# Autodesk Inventor assembly: J005558
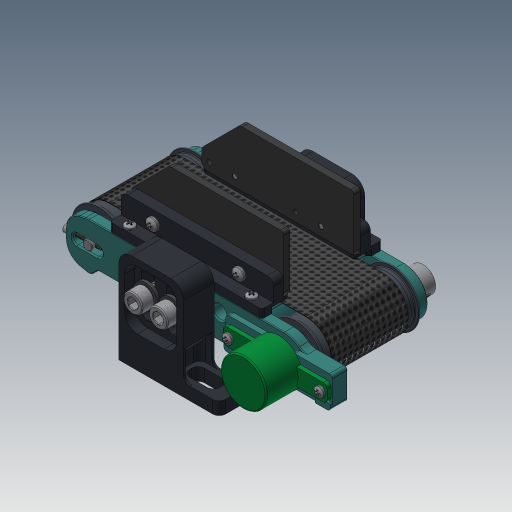
[picture p0: Inventor's stored thumbnail of the model, 512x512]
Saved by Autodesk Inventor 2023.3 (Build 273359000, 359)
## iProperties
Created: 2014-11-17
Vendor: HHMI: JRC - ID&F
Document SubType Name: Assembly
Designer: ARNOLDJ
Description: NRB TREADMILL ASSY
Project: COMMON
Part Number: J005558
RuleStatus: InUse
AfterDocSave0: file://Part Number Cleaner
DESIGN DEPARTMENT: HHMI: JRC - ID&F
LAB/DEPT: COMMON
REQUESTING SCIENTIST: COMMON
SPECIAL FINISH: N/A
SURFACE ROUGHNESS: N/A
ALTERED ITEM PART NUMBER: N/A
ALTERED ITEM VENDOR: N/A
ALTERED ITEM DESCRIPTION: N/A
Revision Number: 0
## Documents named in this file (27)
- C:\_WORKSPACE\DATA\PROJECTS\TREADMILLS\MOUSE NARROW RIBBON BELT TREADMILL\MCAD\NRB DRIVEN TREADMILL ASSY.iam
- C:\_WORKSPACE\DATA\PROJECTS\TREADMILLS\MOUSE MOTOR DRIVEN TREADMILL\MCAD\90107A126.ipt
- C:\_WORKSPACE\DATA\PROJECTS\TREADMILLS\MOUSE MOTOR DRIVEN TREADMILL\MCAD\57155K335.ipt
- C:\_WORKSPACE\DATA\PROJECTS\TREADMILLS\MOUSE MOTOR DRIVEN TREADMILL\MCAD\R233-05-5.ipt
- C:\_WORKSPACE\DATA\PROJECTS\TREADMILLS\MOUSE WIDE RIBBON BELT TREADMILL\MCAD\HEDR-5420-ES214.ipt
- C:\_WORKSPACE\DATA\PROJECTS\TREADMILLS\MOUSE NARROW RIBBON BELT TREADMILL\MCAD\NRB ROLLER.ipt
- C:\_WORKSPACE\DATA\PROJECTS\TREADMILLS\MOUSE NARROW RIBBON BELT TREADMILL\MCAD\NRB DRIVE ROLLER.ipt
- C:\_WORKSPACE\DATA\PROJECTS\TREADMILLS\MOUSE NARROW RIBBON BELT TREADMILL\MCAD\NRB IDLER SHAFT.ipt
- C:\_WORKSPACE\DATA\PROJECTS\TREADMILLS\MOUSE NARROW RIBBON BELT TREADMILL\MCAD\NRB DRIVE SHAFT.ipt
- C:\_WORKSPACE\DATA\PROJECTS\TREADMILLS\MOUSE NARROW RIBBON BELT TREADMILL\MCAD\98317A214.ipt
- C:\_WORKSPACE\DATA\PROJECTS\TREADMILLS\MOUSE NARROW RIBBON BELT TREADMILL\MCAD\57155K336.ipt
- C:\_WORKSPACE\DATA\PROJECTS\TREADMILLS\MOUSE NARROW RIBBON BELT TREADMILL\MCAD\9946K110.ipt
- C:\_WORKSPACE\DATA\PROJECTS\TREADMILLS\MOUSE NARROW RIBBON BELT TREADMILL\MCAD\NRB BRKT SIDE WALL.ipt
- C:\_WORKSPACE\DATA\PROJECTS\TREADMILLS\MOUSE NARROW RIBBON BELT TREADMILL\MCAD\92290A746.ipt
- C:\_WORKSPACE\DATA\PROJECTS\TREADMILLS\TREADMILL LEGO\MCAD\ROLLING WHEEL TYPE\90965A170.ipt
- C:\_WORKSPACE\DATA\PROJECTS\TREADMILLS\TREADMILL LEGO\MCAD\ROLLING WHEEL TYPE\92196A540.ipt
- C:\_WORKSPACE\DATA\PROJECTS\TREADMILLS\MOUSE NARROW RIBBON BELT TREADMILL\MCAD\NRB ADJ BRKT MR.ipt
- C:\_WORKSPACE\DATA\PROJECTS\TREADMILLS\MOUSE NARROW RIBBON BELT TREADMILL\MCAD\NRB ADJ BRKT ML.ipt
- C:\_WORKSPACE\DATA\PROJECTS\TREADMILLS\MOUSE NARROW RIBBON BELT TREADMILL\MCAD\NRB BELT.ipt
- C:\_WORKSPACE\DATA\PROJECTS\TREADMILLS\MOUSE NARROW RIBBON BELT TREADMILL\MCAD\92000A118.ipt
- C:\_WORKSPACE\DATA\PROJECTS\TREADMILLS\MOUSE NARROW RIBBON BELT TREADMILL\MCAD\NRB MAIN BODY INSERTS.ipt
- C:\_WORKSPACE\DATA\PROJECTS\TREADMILLS\MOUSE NARROW RIBBON BELT TREADMILL\MCAD\94785A415_TYPE 18-8 STAINLESS STEEL SQUARE NUT.ipt
- C:\_WORKSPACE\DATA\PROJECTS\TREADMILLS\MOUSE NARROW RIBBON BELT TREADMILL\MCAD\NRB LOW GUIDE RAIL INSERTS.ipt
- C:\_WORKSPACE\DATA\PROJECTS\TREADMILLS\MOUSE NARROW RIBBON BELT TREADMILL\MCAD\91828A113_TYPE 18-8 STAINLESS STEEL HEX NUT.ipt
- C:\_WORKSPACE\DATA\COMMON\McMaster\92000A106.ipt
- C:\_WORKSPACE\DATA\COMMON\McMaster\92000A112.ipt
- C:\_WORKSPACE\DATA\PROJECTS\TREADMILLS\MOUSE NARROW RIBBON BELT TREADMILL\MCAD\HEDR-5420-ES214_DISC.ipt
## Components (53 placed, 26 different names)
1. NRB MAIN BODY INSERTS:1 — Mate:11, Mate:12, Mate:78, Mate:79, Mate:80, Mate:81, Mate:97, Mate:99, Mate:124, Mate:125, Mate:126, Mate:127, Mate:179, Mate:180, Mate:181, Mate:185, Mate:186, Mate:187, Mate:211, Mate:212, Mate:213, Mate:214, Mate:215, Mate:216, Mate:217, Mate:218, Mate:219, Mate:220, Mate:221, Mate:222, Mate:223, Mate:224, Angle:7, Angle:8, Angle:9, Mate:225, Mate:226, Angle:10, Mate:227, Mate:228, Mate:229
2. 57155K336:2 — Mate:11, Mate:12, Mate:126, Mate:127
3. 57155K336:1 — Mate:124, Mate:125
4. NRB ROLLER:1 — Mate:18, Mate:19, Mate:35, Flush:5, Mate:54, Mate:55, Mate:56, Mate:57
5. 57155K335:7 — Mate:56, Mate:57
6. 57155K335:8 — Mate:54, Mate:55
7. NRB IDLER SHAFT:1 — Flush:2, Mate:35, Angle:5
8. NRB DRIVE SHAFT:1 — Mate:94, Mate:98, Mate:243, Flush:6
9. 9946K110:1
10. NRB DRIVE ROLLER:1 — Mate:60
11. NRB BELT:1 — Mate:62, Mate:63, Angle:6
12. 90107A126:1 — Mate:78, Mate:79
13. 90107A126:2 — Mate:80, Mate:81
14. 92290A746:1
15. 92290A746:2
16. R233-05-5:1
17. 98317A214:1
18. HEDR-5420-ES214:1 — Mate:97, Mate:98, Mate:99, Mate:231, Mate:232, Mate:241, Mate:242
19. 92196A540:3 — Mate:230
20. 90965A170:1
21. 92196A540:4
22. 90965A170:2
23. NRB ADJ BRKT ML:1
24. NRB ADJ BRKT MR:1
25. 92196A540:2
26. 90965A170:4
27. 92196A540:1
28. 90965A170:3
29. 92000A112:1 — Mate:233, Mate:234
30. 92000A112:2 — Mate:235, Mate:236
31. 92000A112:3 — Mate:237, Mate:238
32. 92000A112:4 — Mate:239, Mate:240
33. 92000A118:1 — Mate:193, Mate:194
34. 92000A118:2 — Mate:191, Mate:192
35. 92000A118:3 — Mate:207, Mate:208
36. 92000A118:4 — Mate:205, Mate:206
37. NRB LOW GUIDE RAIL INSERTS:1 — Mate:179, Mate:180, Mate:181, Mate:182, Mate:183, Mate:184, Mate:205, Mate:206, Mate:207, Mate:208, Mate:237, Mate:238, Mate:239, Mate:240
38. NRB BRKT SIDE WALL:2 — Mate:188, Mate:189, Mate:190, Mate:192
39. NRB BRKT SIDE WALL:3 — Mate:182, Mate:183, Mate:184
40. NRB LOW GUIDE RAIL INSERTS:2 — Mate:185, Mate:186, Mate:187, Mate:188, Mate:189, Mate:190, Mate:191, Mate:193, Mate:194, Mate:233, Mate:234, Mate:235, Mate:236
41. 94785A415_TYPE 18-8 STAINLESS STEEL SQUARE NUT:1 — Mate:211, Mate:212
42. 94785A415_TYPE 18-8 STAINLESS STEEL SQUARE NUT:2 — Mate:213, Mate:214
43. 91828A113_TYPE 18-8 STAINLESS STEEL HEX NUT:1 — Mate:215, Mate:216
44. 91828A113_TYPE 18-8 STAINLESS STEEL HEX NUT:2 — Mate:217, Mate:218
45. 91828A113_TYPE 18-8 STAINLESS STEEL HEX NUT:3 — Mate:219, Mate:220, Angle:8
46. 91828A113_TYPE 18-8 STAINLESS STEEL HEX NUT:4 — Mate:221, Mate:222, Angle:9
47. 91828A113_TYPE 18-8 STAINLESS STEEL HEX NUT:5 — Mate:223, Mate:224, Angle:7
48. 91828A113_TYPE 18-8 STAINLESS STEEL HEX NUT:6 — Mate:225, Mate:226, Angle:10
49. 94785A415_TYPE 18-8 STAINLESS STEEL SQUARE NUT:3 — Mate:227, Mate:228
50. 94785A415_TYPE 18-8 STAINLESS STEEL SQUARE NUT:4 — Mate:229, Mate:230
51. 92000A106:1 — Mate:231, Mate:232
52. 92000A112:5 — Mate:241, Mate:242
53. HEDR-5420-ES214_DISC:1 — Mate:243, Flush:6
## Relationships (129: Mate 119, Angle 6, Flush 4)
- Mate:11: NRB MAIN BODY INSERTS:1 ↔ 57155K336:2
- Mate:12: NRB MAIN BODY INSERTS:1 ↔ 57155K336:2
- Flush:1
- Mate:15
- Mate:16
- Mate:18: NRB ROLLER:1
- Mate:19: NRB ROLLER:1
- Flush:2: NRB IDLER SHAFT:1
- Mate:35: NRB ROLLER:1 ↔ NRB IDLER SHAFT:1
- Mate:94: NRB DRIVE SHAFT:1
- [Mate]: 57155K336:2 ↔ 9946K110:1
- [Mate]: NRB DRIVE SHAFT:1 ↔ 9946K110:1
- Flush:5: NRB ROLLER:1
- Mate:54: NRB ROLLER:1 ↔ 57155K335:8
- Mate:55: NRB ROLLER:1 ↔ 57155K335:8
- Mate:56: NRB ROLLER:1 ↔ 57155K335:7
- Mate:57: NRB ROLLER:1 ↔ 57155K335:7
- Angle:5 (0 deg): NRB IDLER SHAFT:1
- Mate:60: NRB DRIVE ROLLER:1
- Mate:62: NRB BELT:1
- Mate:63: NRB BELT:1
- Angle:6 (180 deg): NRB BELT:1
- Mate:78: NRB MAIN BODY INSERTS:1 ↔ 90107A126:1
- Mate:79: NRB MAIN BODY INSERTS:1 ↔ 90107A126:1
- Mate:80: NRB MAIN BODY INSERTS:1 ↔ 90107A126:2
- Mate:81: NRB MAIN BODY INSERTS:1 ↔ 90107A126:2
- [Mate]: 90107A126:2 ↔ 92290A746:1
- [Mate]: NRB MAIN BODY INSERTS:1 ↔ 92290A746:1
- [Mate]: 90107A126:1 ↔ 92290A746:2
- [Mate]: NRB MAIN BODY INSERTS:1 ↔ 92290A746:2
- [Mate]: NRB MAIN BODY INSERTS:1 ↔ 57155K336:1
- [Mate]: NRB MAIN BODY INSERTS:1 ↔ 57155K336:1
- [Mate]: 57155K336:2 ↔ 9946K110:1
- [Mate]: NRB DRIVE SHAFT:1 ↔ 98317A214:1
- [Mate]: NRB DRIVE SHAFT:1 ↔ 98317A214:1
- Mate:97: NRB MAIN BODY INSERTS:1 ↔ HEDR-5420-ES214:1
- Mate:98: NRB DRIVE SHAFT:1 ↔ HEDR-5420-ES214:1
- Mate:99: NRB MAIN BODY INSERTS:1 ↔ HEDR-5420-ES214:1
- Mate:124: NRB MAIN BODY INSERTS:1 ↔ 57155K336:1
- Mate:125: NRB MAIN BODY INSERTS:1 ↔ 57155K336:1
- Mate:126: NRB MAIN BODY INSERTS:1 ↔ 57155K336:2
- Mate:127: NRB MAIN BODY INSERTS:1 ↔ 57155K336:2
- [Mate]: NRB MAIN BODY INSERTS:1 ↔ NRB ADJ BRKT MR:1
- [Mate]: NRB MAIN BODY INSERTS:1 ↔ NRB ADJ BRKT MR:1
- [Mate]: NRB MAIN BODY INSERTS:1 ↔ NRB ADJ BRKT ML:1
- [Mate]: NRB MAIN BODY INSERTS:1 ↔ NRB ADJ BRKT ML:1
- [Mate]: NRB MAIN BODY INSERTS:1 ↔ NRB ADJ BRKT MR:1
- [Mate]: NRB ADJ BRKT MR:1 ↔ 90965A170:3
- [Mate]: NRB MAIN BODY INSERTS:1 ↔ 90965A170:3
- [Mate]: 92196A540:1 ↔ 90965A170:3
- [Mate]: NRB MAIN BODY INSERTS:1 ↔ 92196A540:1
- [Mate]: NRB ADJ BRKT MR:1 ↔ 90965A170:4
- [Mate]: NRB MAIN BODY INSERTS:1 ↔ 90965A170:4
- [Mate]: 92196A540:2 ↔ 90965A170:4
- [Mate]: 92196A540:2 ↔ 90965A170:4
- [Mate]: 90965A170:2 ↔ NRB ADJ BRKT ML:1
- [Mate]: NRB MAIN BODY INSERTS:1 ↔ 90965A170:2
- [Mate]: 90965A170:1 ↔ NRB ADJ BRKT ML:1
- [Mate]: NRB MAIN BODY INSERTS:1 ↔ 90965A170:1
- [Mate]: 92196A540:4 ↔ 90965A170:2
- [Mate]: 92196A540:4 ↔ 90965A170:2
- [Mate]: 92196A540:3 ↔ 90965A170:1
- [Mate]: 92196A540:3 ↔ 90965A170:1
- Mate:179: NRB MAIN BODY INSERTS:1 ↔ NRB LOW GUIDE RAIL INSERTS:1
- Mate:180: NRB MAIN BODY INSERTS:1 ↔ NRB LOW GUIDE RAIL INSERTS:1
- Mate:181: NRB MAIN BODY INSERTS:1 ↔ NRB LOW GUIDE RAIL INSERTS:1
- Mate:182: NRB LOW GUIDE RAIL INSERTS:1 ↔ NRB BRKT SIDE WALL:3
- Mate:183: NRB LOW GUIDE RAIL INSERTS:1 ↔ NRB BRKT SIDE WALL:3
- Mate:184: NRB LOW GUIDE RAIL INSERTS:1 ↔ NRB BRKT SIDE WALL:3
- Mate:185: NRB MAIN BODY INSERTS:1 ↔ NRB LOW GUIDE RAIL INSERTS:2
- Mate:186: NRB MAIN BODY INSERTS:1 ↔ NRB LOW GUIDE RAIL INSERTS:2
- Mate:187: NRB MAIN BODY INSERTS:1 ↔ NRB LOW GUIDE RAIL INSERTS:2
- Mate:188: NRB BRKT SIDE WALL:2 ↔ NRB LOW GUIDE RAIL INSERTS:2
- Mate:189: NRB BRKT SIDE WALL:2 ↔ NRB LOW GUIDE RAIL INSERTS:2
- Mate:190: NRB BRKT SIDE WALL:2 ↔ NRB LOW GUIDE RAIL INSERTS:2
- Mate:191: 92000A118:2 ↔ NRB LOW GUIDE RAIL INSERTS:2
- Mate:192: 92000A118:2 ↔ NRB BRKT SIDE WALL:2
- Mate:193: 92000A118:1 ↔ NRB LOW GUIDE RAIL INSERTS:2
- Mate:194: 92000A118:1 ↔ NRB LOW GUIDE RAIL INSERTS:2
- [Mate]: 92000A112:1 ↔ NRB LOW GUIDE RAIL INSERTS:2
- [Mate]: 92000A112:1 ↔ NRB LOW GUIDE RAIL INSERTS:2
- [Mate]: 92000A112:2 ↔ NRB LOW GUIDE RAIL INSERTS:2
- [Mate]: 92000A112:2 ↔ NRB LOW GUIDE RAIL INSERTS:2
- [Mate]: 92000A112:3 ↔ NRB LOW GUIDE RAIL INSERTS:1
- [Mate]: 92000A112:3 ↔ NRB LOW GUIDE RAIL INSERTS:1
- Mate:205: 92000A118:4 ↔ NRB LOW GUIDE RAIL INSERTS:1
- Mate:206: 92000A118:4 ↔ NRB LOW GUIDE RAIL INSERTS:1
- Mate:207: 92000A118:3 ↔ NRB LOW GUIDE RAIL INSERTS:1
- Mate:208: 92000A118:3 ↔ NRB LOW GUIDE RAIL INSERTS:1
- [Mate]: 92000A112:4 ↔ NRB LOW GUIDE RAIL INSERTS:1
- [Mate]: 92000A112:4 ↔ NRB LOW GUIDE RAIL INSERTS:1
- Mate:211: NRB MAIN BODY INSERTS:1 ↔ 94785A415_TYPE 18-8 STAINLESS STEEL SQUARE NUT:1
- Mate:212: NRB MAIN BODY INSERTS:1 ↔ 94785A415_TYPE 18-8 STAINLESS STEEL SQUARE NUT:1
- Mate:213: NRB MAIN BODY INSERTS:1 ↔ 94785A415_TYPE 18-8 STAINLESS STEEL SQUARE NUT:2
- Mate:214: NRB MAIN BODY INSERTS:1 ↔ 94785A415_TYPE 18-8 STAINLESS STEEL SQUARE NUT:2
- Mate:215: NRB MAIN BODY INSERTS:1 ↔ 91828A113_TYPE 18-8 STAINLESS STEEL HEX NUT:1
- Mate:216: NRB MAIN BODY INSERTS:1 ↔ 91828A113_TYPE 18-8 STAINLESS STEEL HEX NUT:1
- Mate:217: NRB MAIN BODY INSERTS:1 ↔ 91828A113_TYPE 18-8 STAINLESS STEEL HEX NUT:2
- Mate:218: NRB MAIN BODY INSERTS:1 ↔ 91828A113_TYPE 18-8 STAINLESS STEEL HEX NUT:2
- Mate:219: NRB MAIN BODY INSERTS:1 ↔ 91828A113_TYPE 18-8 STAINLESS STEEL HEX NUT:3
- Mate:220: NRB MAIN BODY INSERTS:1 ↔ 91828A113_TYPE 18-8 STAINLESS STEEL HEX NUT:3
- Mate:221: NRB MAIN BODY INSERTS:1 ↔ 91828A113_TYPE 18-8 STAINLESS STEEL HEX NUT:4
- Mate:222: NRB MAIN BODY INSERTS:1 ↔ 91828A113_TYPE 18-8 STAINLESS STEEL HEX NUT:4
- Mate:223: NRB MAIN BODY INSERTS:1 ↔ 91828A113_TYPE 18-8 STAINLESS STEEL HEX NUT:5
- Mate:224: NRB MAIN BODY INSERTS:1 ↔ 91828A113_TYPE 18-8 STAINLESS STEEL HEX NUT:5
- Angle:7 (0 deg): NRB MAIN BODY INSERTS:1 ↔ 91828A113_TYPE 18-8 STAINLESS STEEL HEX NUT:5
- Angle:8 (0 deg): NRB MAIN BODY INSERTS:1 ↔ 91828A113_TYPE 18-8 STAINLESS STEEL HEX NUT:3
- Angle:9 (0 deg): NRB MAIN BODY INSERTS:1 ↔ 91828A113_TYPE 18-8 STAINLESS STEEL HEX NUT:4
- Mate:225: NRB MAIN BODY INSERTS:1 ↔ 91828A113_TYPE 18-8 STAINLESS STEEL HEX NUT:6
- Mate:226: NRB MAIN BODY INSERTS:1 ↔ 91828A113_TYPE 18-8 STAINLESS STEEL HEX NUT:6
- Angle:10 (0 deg): NRB MAIN BODY INSERTS:1 ↔ 91828A113_TYPE 18-8 STAINLESS STEEL HEX NUT:6
- Mate:227: NRB MAIN BODY INSERTS:1 ↔ 94785A415_TYPE 18-8 STAINLESS STEEL SQUARE NUT:3
- Mate:228: NRB MAIN BODY INSERTS:1 ↔ 94785A415_TYPE 18-8 STAINLESS STEEL SQUARE NUT:3
- Mate:229: NRB MAIN BODY INSERTS:1 ↔ 94785A415_TYPE 18-8 STAINLESS STEEL SQUARE NUT:4
- Mate:230: 92196A540:3 ↔ 94785A415_TYPE 18-8 STAINLESS STEEL SQUARE NUT:4
- Mate:231: HEDR-5420-ES214:1 ↔ 92000A106:1
- Mate:232: HEDR-5420-ES214:1 ↔ 92000A106:1
- Mate:233: 92000A112:1 ↔ NRB LOW GUIDE RAIL INSERTS:2
- Mate:234: 92000A112:1 ↔ NRB LOW GUIDE RAIL INSERTS:2
- Mate:235: 92000A112:2 ↔ NRB LOW GUIDE RAIL INSERTS:2
- Mate:236: 92000A112:2 ↔ NRB LOW GUIDE RAIL INSERTS:2
- Mate:237: 92000A112:3 ↔ NRB LOW GUIDE RAIL INSERTS:1
- Mate:238: 92000A112:3 ↔ NRB LOW GUIDE RAIL INSERTS:1
- Mate:239: 92000A112:4 ↔ NRB LOW GUIDE RAIL INSERTS:1
- Mate:240: 92000A112:4 ↔ NRB LOW GUIDE RAIL INSERTS:1
- Mate:241: HEDR-5420-ES214:1 ↔ 92000A112:5
- Mate:242: HEDR-5420-ES214:1 ↔ 92000A112:5
- Mate:243: NRB DRIVE SHAFT:1 ↔ HEDR-5420-ES214_DISC:1
- Flush:6 (-0.508 mm): NRB DRIVE SHAFT:1 ↔ HEDR-5420-ES214_DISC:1
## Named parameters: d171_d110 = 0 mm, d172_d111 = 0 mm, d173_d112 = 0 mm, d174_d113 = 0 mm, d175_d114 = 0 mm, d176_d115 = 0 mm, d177_d116 = 0 mm, d183_d122 = 0 mm, d184_d123 = 0 mm, d185_d124 = 0 mm, d186_d125 = 0 mm
